# Autodesk Inventor assembly: ЛЦМК.30000,00,00,00 СБ Шлем
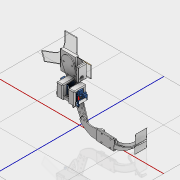
[picture p0: Inventor's stored thumbnail of the model, 180x180]
Saved by Autodesk Inventor 2021.2 (Build 252289000, 289)
## iProperties
Created: 2025-11-22
Part Number: ЛЦМК.30000,00,00,00 СБ Шлем
Document SubType Name: Assembly
Designer: Захаров
Author: Захаров
## Documents named in this file (5)
- C:\Users\User\Documents\Inventor\ЛЦМК.30000.00.00.00 Шлем\ЛЦМК.30000.00.00.00 СБ Шлем.iam
- ЛЦМК.30000.00.00.00 СБ Шлем.iam
- C:\Users\User\Documents\Inventor\ЛЦМК.30000.00.00.00 Шлем\ЛЦМК.30000.10.00.00 Корпус XIAO\ЛЦМК.30000.10.00.00 СБ Корпус XIAO.iam
- C:\Users\User\Documents\Inventor\ЛЦМК.30000.00.00.00 Шлем\ЛЦМК.30000.20.00.00 Держатель OLED\ЛЦМК.30000.20.00.00 СБ Держатель OLED.iam
- C:\Users\User\Documents\Inventor\ЛЦМК.30000.00.00.00 Шлем\ЛЦМК.30000.30.00.00 Крепление\ЛЦМК.30000.30.00.00 СБ Крепление.iam
## Components (3 placed, 3 different names)
1. ЛЦМК.30000.10.00.00 СБ Корпус XIAO:1 [sub-assembly] — Вставка:2, Вставка:3
2. ЛЦМК.30000.20.00.00 СБ Держатель OLED:1 [sub-assembly] — Вставка:1, Угол:1
3. ЛЦМК.30000.30.00.00 СБ Крепление:1 [sub-assembly] — Вставка:1, Угол:1, Вставка:2, Вставка:3
## Relationships (4: Insert 3, Angle 1)
- Вставка:1 [Insert]: ЛЦМК.30000.20.00.00 СБ Держатель OLED:1 ↔ ЛЦМК.30000.30.00.00 СБ Крепление:1
- Угол:1 [Angle] (70 deg): ЛЦМК.30000.20.00.00 СБ Держатель OLED:1 ↔ ЛЦМК.30000.30.00.00 СБ Крепление:1
- Вставка:2 [Insert]: ЛЦМК.30000.10.00.00 СБ Корпус XIAO:1 ↔ ЛЦМК.30000.30.00.00 СБ Крепление:1
- Вставка:3 [Insert]: ЛЦМК.30000.10.00.00 СБ Корпус XIAO:1 ↔ ЛЦМК.30000.30.00.00 СБ Крепление:1
